# Autodesk Inventor assembly: scara
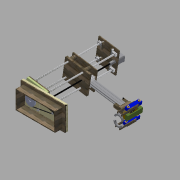
[picture p0: Inventor's stored thumbnail of the model, 180x180]
Saved by Autodesk Inventor 2019 (Build 230136000, 136)
## iProperties
Created: 2021-11-05
Part Number: scara
Document SubType Name: Assembly
Designer: Mohamed
Author: Mohamed
## Documents named in this file (9)
- F:\Semester 7\Design of mechatronics 1\SSCARA Robot\scara.iam
- F:\Semester 7\Design of mechatronics 1\SSCARA Robot\elevator.iam
- F:\Semester 7\Design of mechatronics 1\SSCARA Robot\Griper_v slot.iam
- F:\Semester 7\Design of mechatronics 1\SSCARA Robot\Tower.iam
- F:\Semester 7\Design of mechatronics 1\SSCARA Robot\Base 2.0.iam
- F:\Semester 7\Design of mechatronics 1\SSCARA Robot\b_base_table.ipt
- F:\Semester 7\Design of mechatronics 1\SSCARA Robot\idler pulley.ipt
- F:\Semester 7\Design of mechatronics 1\SSCARA Robot\idler puley bolt.ipt
- F:\Semester 7\Design of mechatronics 1\SSCARA Robot\110 teeth gt2 pulley.ipt
## Components (8 placed, 8 different names)
1. elevator:1 [sub-assembly] — Mate:1, Mate:2, Mate:3, Mate:4, Mate:5
2. Griper_v slot:1 [sub-assembly] — Mate:1, Mate:2, Mate:3
3. Tower:1 [sub-assembly] — Mate:4, Mate:5, Mate:13, Mate:14, Mate:15
4. Base 2.0:1 [sub-assembly] — Mate:7, Tangent:1, Tangent:2, Mate:8, Mate:9, Mate:12
5. b_base_table:1 — Mate:10, Mate:11, Mate:12, Mate:13, Mate:14, Mate:15
6. idler pulley:1 — Mate:6, Tangent:2
7. idler puley bolt:1 — Mate:6, Mate:7, Tangent:1
8. 110 teeth gt2 pulley:1 — Mate:8, Mate:9, Mate:10, Mate:11
## Relationships (17: Mate 15, Tangent 2)
- Mate:1: elevator:1 ↔ Griper_v slot:1
- Mate:2: elevator:1 ↔ Griper_v slot:1
- Mate:3: elevator:1 ↔ Griper_v slot:1
- Mate:4: elevator:1 ↔ Tower:1
- Mate:5: elevator:1 ↔ Tower:1
- Mate:6: idler pulley:1 ↔ idler puley bolt:1
- Mate:7: Base 2.0:1 ↔ idler puley bolt:1
- Tangent:1: Base 2.0:1 ↔ idler puley bolt:1
- Tangent:2: Base 2.0:1 ↔ idler pulley:1
- Mate:8: Base 2.0:1 ↔ 110 teeth gt2 pulley:1
- Mate:9: Base 2.0:1 ↔ 110 teeth gt2 pulley:1
- Mate:10: b_base_table:1 ↔ 110 teeth gt2 pulley:1
- Mate:11: b_base_table:1 ↔ 110 teeth gt2 pulley:1
- Mate:12: Base 2.0:1 ↔ b_base_table:1
- Mate:13: Tower:1 ↔ b_base_table:1
- Mate:14: Tower:1 ↔ b_base_table:1
- Mate:15: Tower:1 ↔ b_base_table:1
